# Autodesk Inventor assembly: Assembly w Phone Exploded
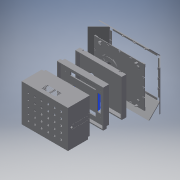
[picture p0: Inventor's stored thumbnail of the model, 180x180]
Saved by Autodesk Inventor 2017 (Build 210142000, 142)
## iProperties
Created: 2018-02-08
Part Number: Assembly w Phone Exploded
Document SubType Name: Assembly
Designer: Arjuna
Author: Arjuna
## Documents named in this file (9)
- D:\Users\Arjuna\Documents\NTU\FYP\Hardware\Assembly w Phone Exploded.iam
- D:\Users\Arjuna\Documents\NTU\FYP\Hardware\Bottom Roof.ipt
- D:\Users\Arjuna\Documents\NTU\FYP\Hardware\Bottom Assembly.iam
- D:\Users\Arjuna\Documents\NTU\FYP\Hardware\Platform Assembly.iam
- D:\Users\Arjuna\Documents\NTU\FYP\Hardware\Top Roof Assembly.iam
- D:\Users\Arjuna\Documents\NTU\FYP\Hardware\Roof Length Extension.ipt
- D:\Users\Arjuna\Documents\NTU\FYP\Hardware\Roof Width Extension.ipt
- D:\Users\Arjuna\Documents\NTU\FYP\Hardware\Phone.ipt
- D:\Users\Arjuna\Documents\NTU\FYP\Hardware\Lens.ipt
## Components (10 placed, 8 different names)
1. Bottom Assembly:1 [sub-assembly] — Flush:1, Flush:2, Flush:3, Flush:4, Flush:5, Flush:6, Flush:7, Flush:8, Flush:9, Mate:1
2. Platform Assembly:1 [sub-assembly] — Flush:4, Flush:5, Mate:1, Mate:2, Flush:13, Mate:21
3. Bottom Roof:1 — Flush:6, Flush:7, Mate:2, Mate:3
4. Top Roof Assembly:1 [sub-assembly] — Flush:8, Flush:9, Mate:3, Mate:11, Mate:12, Mate:13, Mate:14, Mate:15, Mate:16, Mate:17, Mate:18
5. Roof Length Extension:1 — Mate:6, Mate:13, Mate:16
6. Roof Length Extension:2 — Flush:10, Mate:11, Mate:18
7. Roof Width Extension:1 — Flush:11, Mate:14, Mate:15
8. Roof Width Extension:2 — Mate:5, Mate:12, Mate:17
9. Phone:1 — Mate:19, Flush:12, Mate:20, Flush:13, Mate:21
10. Lens:1 — Mate:19, Flush:12, Mate:20
## Relationships (29: Mate 16, Flush 13)
- Flush:1: Bottom Assembly:1
- Flush:2: Bottom Assembly:1
- Flush:3: Bottom Assembly:1
- Flush:4: Bottom Assembly:1 ↔ Platform Assembly:1
- Flush:5: Bottom Assembly:1 ↔ Platform Assembly:1
- Flush:6: Bottom Assembly:1 ↔ Bottom Roof:1
- Flush:7: Bottom Assembly:1 ↔ Bottom Roof:1
- Flush:8: Bottom Assembly:1 ↔ Top Roof Assembly:1
- Flush:9: Bottom Assembly:1 ↔ Top Roof Assembly:1
- Mate:1 (75 mm): Bottom Assembly:1 ↔ Platform Assembly:1
- Mate:2 (75 mm): Platform Assembly:1 ↔ Bottom Roof:1
- Mate:3 (75 mm): Bottom Roof:1 ↔ Top Roof Assembly:1
- Flush:11: Roof Width Extension:1
- Mate:5: Roof Width Extension:2
- Mate:6: Roof Length Extension:1
- Flush:10: Roof Length Extension:2
- Mate:11 (75 mm): Top Roof Assembly:1 ↔ Roof Length Extension:2
- Mate:12 (75 mm): Top Roof Assembly:1 ↔ Roof Width Extension:2
- Mate:13 (75 mm): Top Roof Assembly:1 ↔ Roof Length Extension:1
- Mate:14 (75 mm): Top Roof Assembly:1 ↔ Roof Width Extension:1
- Mate:15: Top Roof Assembly:1 ↔ Roof Width Extension:1
- Mate:16: Top Roof Assembly:1 ↔ Roof Length Extension:1
- Mate:17: Top Roof Assembly:1 ↔ Roof Width Extension:2
- Mate:18: Top Roof Assembly:1 ↔ Roof Length Extension:2
- Mate:19: Phone:1 ↔ Lens:1
- Flush:12: Phone:1 ↔ Lens:1
- Mate:20: Phone:1 ↔ Lens:1
- Flush:13: Platform Assembly:1 ↔ Phone:1
- Mate:21: Platform Assembly:1 ↔ Phone:1
